# Autodesk Inventor assembly: armsteun links
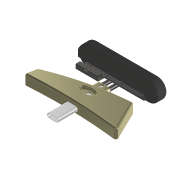
[picture p0: Inventor's stored thumbnail of the model, 180x180]
Saved by Autodesk Inventor 2020.3 (Build 243373000, 373)
## iProperties
Created: 2020-09-11
Part Number: armsteun links
Document SubType Name: Assembly
Designer: Svend
Author: Svend
## Documents named in this file (6)
- C:\Users\Svend\OneDrive\Documents\GitHub\Rolstoel\armsteun links.iam
- C:\Users\Svend\OneDrive\Documents\GitHub\Rolstoel\armsteun.ipt
- C:\Users\Svend\OneDrive\Documents\GitHub\Rolstoel\beugel armsteun.ipt
- C:\Users\Svend\OneDrive\Documents\GitHub\Rolstoel\buis armsteun.ipt
- C:\Users\Svend\OneDrive\Documents\GitHub\Rolstoel\profiel armsteun.ipt
- C:\Users\Svend\OneDrive\Documents\GitHub\Rolstoel\armsteun houder.ipt
## Components (5 placed, 5 different names)
1. armsteun houder:1 — Mate:9, Mate:11, Mate:14, Mate:15
2. armsteun:1 — Mate:1, Mate:2, Mate:3, Angle:2
3. beugel armsteun:1 — Mate:1, Mate:2, Mate:3, Mate:6, Mate:10, Mate:11, Mate:12, Mate:13
4. buis armsteun:1 — Mate:9, Mate:10, Angle:2, Mate:14, Mate:15
5. profiel armsteun:1 — Mate:6, Mate:12, Mate:13
## Relationships (12: Mate 11, Angle 1)
- Mate:1: armsteun:1 ↔ beugel armsteun:1
- Mate:2: armsteun:1 ↔ beugel armsteun:1
- Mate:3: armsteun:1 ↔ beugel armsteun:1
- Mate:6: beugel armsteun:1 ↔ profiel armsteun:1
- Mate:9 (2 mm): armsteun houder:1 ↔ buis armsteun:1
- Mate:10: beugel armsteun:1 ↔ buis armsteun:1
- Mate:11 (50 mm): armsteun houder:1 ↔ beugel armsteun:1
- Mate:12: beugel armsteun:1 ↔ profiel armsteun:1
- Mate:13: beugel armsteun:1 ↔ profiel armsteun:1
- Angle:2 (0 deg): armsteun:1 ↔ buis armsteun:1
- Mate:14: armsteun houder:1 ↔ buis armsteun:1
- Mate:15: armsteun houder:1 ↔ buis armsteun:1
